# Autodesk Inventor assembly: YEndstopAssembly
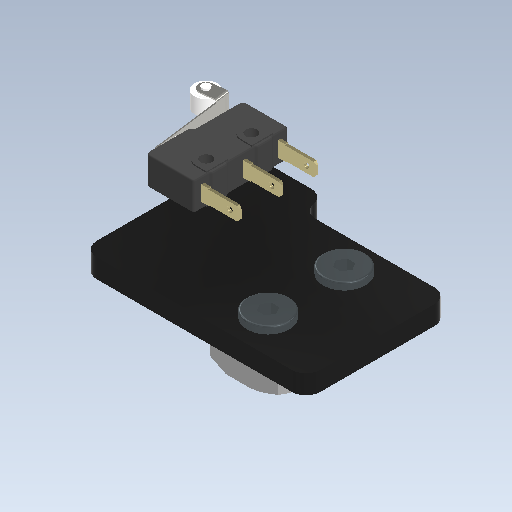
[picture p0: Inventor's stored thumbnail of the model, 512x512]
Saved by Autodesk Inventor 2020.2 (Build 242310000, 310)
## iProperties
Created: 2020-08-28
Part Number: YEndstopAssembly
Document SubType Name: Assembly
Designer: JK
Author: JK
## Documents named in this file (5)
- C:\Users\JK\Documents\Inventor\Anet Upgrade\YEndstopAssembly.iam
- C:\Users\JK\Documents\Inventor\Anet Upgrade\YEndstopMount.ipt
- C:\Users\JK\Documents\Inventor\Anet Upgrade\EndStop.ipt
- C:\Users\JK\Documents\Inventor\Anet Upgrade\M5x12BoltFlatHead.ipt
- C:\Users\JK\Documents\Inventor\Anet Upgrade\T_Slot_Nut_Dropin_3030m5ipt.ipt
## Components (6 placed, 4 different names)
1. YEndstopMount:1 — Mate:1, Mate:2, Angle:1, Mate:3, Mate:4, Mate:5, Angle:2, Mate:8
2. EndStop:1 — Mate:1, Mate:2, Angle:1
3. M5x12BoltFlatHead:1 — Mate:3, Flush:1, Mate:5, Mate:6
4. M5x12BoltFlatHead:2 — Mate:4, Flush:1, Mate:7
5. T_Slot_Nut_Dropin_3030m5ipt:1 — Mate:6, Angle:2, Angle:3, Flush:2, Mate:8
6. T_Slot_Nut_Dropin_3030m5ipt:2 — Mate:7, Angle:3, Flush:2
## Relationships (13: Mate 8, Angle 3, Flush 2)
- Mate:1: YEndstopMount:1 ↔ EndStop:1
- Mate:2: YEndstopMount:1 ↔ EndStop:1
- Angle:1 (0 deg): YEndstopMount:1 ↔ EndStop:1
- Mate:3: YEndstopMount:1 ↔ M5x12BoltFlatHead:1
- Mate:4: YEndstopMount:1 ↔ M5x12BoltFlatHead:2
- Flush:1: M5x12BoltFlatHead:1 ↔ M5x12BoltFlatHead:2
- Mate:5: YEndstopMount:1 ↔ M5x12BoltFlatHead:1
- Mate:6: M5x12BoltFlatHead:1 ↔ T_Slot_Nut_Dropin_3030m5ipt:1
- Mate:7: M5x12BoltFlatHead:2 ↔ T_Slot_Nut_Dropin_3030m5ipt:2
- Angle:2 (0 deg): YEndstopMount:1 ↔ T_Slot_Nut_Dropin_3030m5ipt:1
- Angle:3 (0 deg): T_Slot_Nut_Dropin_3030m5ipt:1 ↔ T_Slot_Nut_Dropin_3030m5ipt:2
- Flush:2: T_Slot_Nut_Dropin_3030m5ipt:1 ↔ T_Slot_Nut_Dropin_3030m5ipt:2
- Mate:8: YEndstopMount:1 ↔ T_Slot_Nut_Dropin_3030m5ipt:1
